# Autodesk Inventor assembly: Intake Assembly
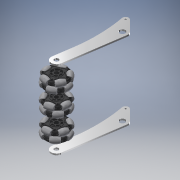
[picture p0: Inventor's stored thumbnail of the model, 180x180]
Saved by Autodesk Inventor 2019.4 (Build 234330000, 330)
## iProperties
Created: 2020-01-28
Part Number: Intake Assembly
Document SubType Name: Assembly
Designer: admin
Author: admin
## Documents named in this file (3)
- C:\Users\admin\Desktop\FRC 2020 Engineering\GitHub\7738-2020\Robot V2\Intake V2\Intake Assembly.iam
- C:\Users\admin\Desktop\FRC 2020 Engineering\GitHub\7738-2020\Robot V2\Intake V2\Intake Arm.ipt
- C:\Users\admin\Desktop\FRC 2020 Engineering\GitHub\7738-2020\Robot V2\Intake V2\Omni Wheel\3_25_Omni-Directional_Wheel_217-4775.iam
## Components (5 placed, 2 different names)
1. Intake Arm:1 — Mate:1, Mate:2, Mate:3, Mate:4, Mate:5, Mate:6, Mate:7
2. Intake Arm:2 — Mate:1, Mate:2, Mate:3, Mate:8
3. 3_25_Omni-Directional_Wheel_217-4775:1 [sub-assembly] — Mate:4
4. 3_25_Omni-Directional_Wheel_217-4775:2 [sub-assembly] — Mate:5
5. 3_25_Omni-Directional_Wheel_217-4775:3 [sub-assembly] — Mate:6
## Relationships (8: Mate 8)
- Mate:1: Intake Arm:1 ↔ Intake Arm:2
- Mate:2: Intake Arm:1 ↔ Intake Arm:2
- Mate:3 (248.6 mm): Intake Arm:1 ↔ Intake Arm:2
- Mate:4: Intake Arm:1 ↔ 3_25_Omni-Directional_Wheel_217-4775:1
- Mate:5: Intake Arm:1 ↔ 3_25_Omni-Directional_Wheel_217-4775:2
- Mate:6: Intake Arm:1 ↔ 3_25_Omni-Directional_Wheel_217-4775:3
- Mate:7: Intake Arm:1
- Mate:8 (119.3 mm): Intake Arm:2
